# Autodesk Inventor assembly: Full Mechanism Assembly
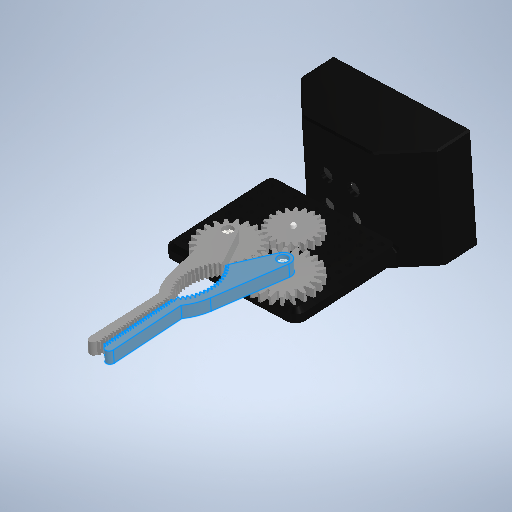
[picture p0: Inventor's stored thumbnail of the model, 512x512]
Saved by Autodesk Inventor 2026.1 (Build 301233000, 233)
## iProperties
Created: 2025-07-17
Part Number: Full Mechanism Assembly
Document SubType Name: Assembly
Designer: AdminForWorker
Title: End Effector Platform v38
Author: AdminForWorker
## Documents named in this file (15)
- C:\Users\kryst\Downloads\fri-12_FinalAssembly\Full Mechanism Assembly.iam
- C:\Users\kryst\Downloads\fri-12_FinalAssembly\N20 Mini Micro Metall Gear Motor DC 3-6-12V v1 v1.ipt
- C:\Users\kryst\Downloads\fri-12_FinalAssembly\XC-430_idle v3.iam
- C:\Users\kryst\Downloads\fri-12_FinalAssembly\End Effector Platform Base.ipt
- C:\Users\kryst\Downloads\fri-12_FinalAssembly\Quanser QUARC EE Board.ipt
- C:\Users\kryst\Downloads\fri-12_FinalAssembly\End Effector Platform.ipt
- C:\Users\kryst\Downloads\fri-12_FinalAssembly\End Effector Platform Compartment Lid.ipt
- C:\Users\kryst\Downloads\fri-12_FinalAssembly\Gripper Motor Cover.ipt
- C:\Users\kryst\Downloads\fri-12_FinalAssembly\Pinion Gear.ipt
- C:\Users\kryst\Downloads\fri-12_FinalAssembly\Gear 2.ipt
- C:\Users\kryst\Downloads\fri-12_FinalAssembly\Gear 3.ipt
- C:\Users\kryst\Downloads\fri-12_FinalAssembly\gripper_V2.ipt
- C:\Users\kryst\Downloads\fri-12_FinalAssembly\gripper_V2_MIR1.ipt
- C:\Users\kryst\Downloads\fri-12_FinalAssembly\Steel M3x16 Pan Head Screw.ipt
- C:\Users\kryst\Downloads\fri-12_FinalAssembly\Steel M3 Hex Nut.ipt
## Components (16 placed, 12 different names)
1. N20 Mini Micro Metall Gear Motor DC 3-6-12V v1 v1:1 — Flush:3, Mate:8, Mate:9, Mate:10, Mate:11, Mate:12, Mate:14
2. XC-430_idle v3:1 [sub-assembly] — Mate:4, Mate:5, Mate:6
3. End Effector Platform Base:1 — Mate:1, Mate:2, Mate:3, Mate:4, Mate:5, Mate:6, Flush:1, Flush:2, Mate:7, Flush:3, Mate:8, Mate:9
4. Quanser QUARC EE Board:1 — Mate:1, Mate:2, Mate:3
5. End Effector Platform:1 — Mate:10, Mate:11, Mate:12, Mate:13, Flush:4, Flush:5, Mate:15, Mate:16, Mate:17, Mate:18, Mate:19, Angle:1, Angle:2, Insert:3, Insert:4, Angle:3, Angle:4
6. End Effector Platform Compartment Lid:1 — Flush:1, Flush:2, Mate:7
7. Gripper Motor Cover:1 — Mate:13, Flush:4, Flush:5
8. Spur Gear1:1 — Mate:14, Mate:15, Rotation:4
9. Spur Gear1:2 — Mate:18, Mate:19, Rotation:1, Mate:22, Mate:23, Rotation:2, Rotation:4
10. Spur Gear1:3 — Mate:16, Mate:17, Rotation:1, Mate:20, Mate:21, Rotation:3
11. gripper_V2:1 — Mate:20, Mate:21, Rotation:3, Insert:1
12. gripper_V2_MIR1:1 — Mate:22, Mate:23, Rotation:2, Insert:2
13. Steel M3x16 Pan Head Screw:1 — Insert:2, Angle:1
14. Steel M3x16 Pan Head Screw:2 — Insert:1, Angle:2
15. Steel M3 Hex Nut:1 — Insert:3, Angle:4
16. Steel M3 Hex Nut:2 — Insert:4, Angle:3
## Relationships (40: Mate 23, Flush 5, RelateRotation 4, Insert 4, Angle 4)
- Mate:1: End Effector Platform Base:1 ↔ Quanser QUARC EE Board:1
- Mate:2: End Effector Platform Base:1 ↔ Quanser QUARC EE Board:1
- Mate:3: End Effector Platform Base:1 ↔ Quanser QUARC EE Board:1
- Mate:4: XC-430_idle v3:1 ↔ End Effector Platform Base:1
- Mate:5: XC-430_idle v3:1 ↔ End Effector Platform Base:1
- Mate:6: XC-430_idle v3:1 ↔ End Effector Platform Base:1
- Flush:1: End Effector Platform Base:1 ↔ End Effector Platform Compartment Lid:1
- Flush:2: End Effector Platform Base:1 ↔ End Effector Platform Compartment Lid:1
- Mate:7: End Effector Platform Base:1 ↔ End Effector Platform Compartment Lid:1
- Flush:3: N20 Mini Micro Metall Gear Motor DC 3-6-12V v1 v1:1 ↔ End Effector Platform Base:1
- Mate:8 (0.2 mm): N20 Mini Micro Metall Gear Motor DC 3-6-12V v1 v1:1 ↔ End Effector Platform Base:1
- Mate:9 (0.2 mm): N20 Mini Micro Metall Gear Motor DC 3-6-12V v1 v1:1 ↔ End Effector Platform Base:1
- Mate:10: N20 Mini Micro Metall Gear Motor DC 3-6-12V v1 v1:1 ↔ End Effector Platform:1
- Mate:11: N20 Mini Micro Metall Gear Motor DC 3-6-12V v1 v1:1 ↔ End Effector Platform:1
- Mate:12: N20 Mini Micro Metall Gear Motor DC 3-6-12V v1 v1:1 ↔ End Effector Platform:1
- Mate:13: End Effector Platform:1 ↔ Gripper Motor Cover:1
- Flush:4: End Effector Platform:1 ↔ Gripper Motor Cover:1
- Flush:5: End Effector Platform:1 ↔ Gripper Motor Cover:1
- Mate:14: N20 Mini Micro Metall Gear Motor DC 3-6-12V v1 v1:1 ↔ Spur Gear1:1
- Mate:15 (5 mm): End Effector Platform:1 ↔ Spur Gear1:1
- Mate:16: End Effector Platform:1 ↔ Spur Gear1:3
- Mate:17: End Effector Platform:1 ↔ Spur Gear1:3
- Mate:18: End Effector Platform:1 ↔ Spur Gear1:2
- Mate:19: End Effector Platform:1 ↔ Spur Gear1:2
- Rotation:1 [RelateRotation] (1 ul): Spur Gear1:2 ↔ Spur Gear1:3
- Mate:20: Spur Gear1:3 ↔ gripper_V2:1
- Mate:21: Spur Gear1:3 ↔ gripper_V2:1
- Mate:22: Spur Gear1:2 ↔ gripper_V2_MIR1:1
- Mate:23: Spur Gear1:2 ↔ gripper_V2_MIR1:1
- Rotation:2 [RelateRotation] (1.912 ul): Spur Gear1:2 ↔ gripper_V2_MIR1:1
- Rotation:3 [RelateRotation] (1.912 ul): Spur Gear1:3 ↔ gripper_V2:1
- Rotation:4 [RelateRotation] (1 ul): Spur Gear1:1 ↔ Spur Gear1:2
- Insert:1: gripper_V2:1 ↔ Steel M3x16 Pan Head Screw:2
- Insert:2: gripper_V2_MIR1:1 ↔ Steel M3x16 Pan Head Screw:1
- Angle:1 (0 deg): End Effector Platform:1 ↔ Steel M3x16 Pan Head Screw:1
- Angle:2 (0 deg): End Effector Platform:1 ↔ Steel M3x16 Pan Head Screw:2
- Insert:3: End Effector Platform:1 ↔ Steel M3 Hex Nut:1
- Insert:4: End Effector Platform:1 ↔ Steel M3 Hex Nut:2
- Angle:3 (0 deg): End Effector Platform:1 ↔ Steel M3 Hex Nut:2
- Angle:4 (0 deg): End Effector Platform:1 ↔ Steel M3 Hex Nut:1
